# Autodesk Inventor assembly: Color Sorter
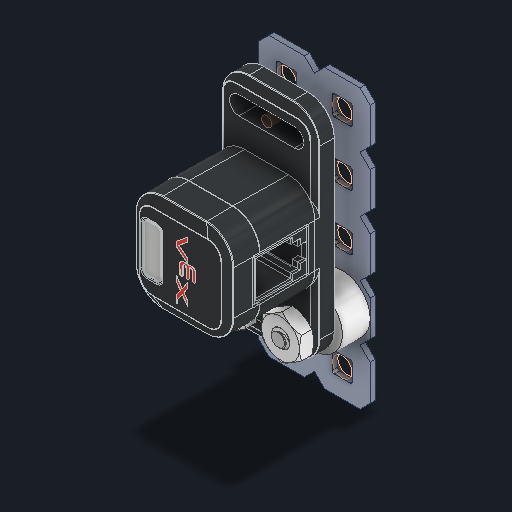
[picture p0: Inventor's stored thumbnail of the model, 512x512]
Saved by Autodesk Inventor 2025.1 (Build 291241000, 241)
## iProperties
Created: 2024-11-18
Part Number: Color Sorter
Document SubType Name: Assembly
Designer: avere
Author: avere
## Documents named in this file (8)
- C:\Users\avere\VEX\High Stakes\CAD\V3\Tower\Color Sorter.iam
- C:\Users\avere\VEX\High Stakes\CAD\ROBOPROS-CAD-Inventor\Electronics\Sensors\V5 Optical Sensor.ipt
- C:\Users\avere\VEX\High Stakes\CAD\ROBOPROS-CAD-Inventor\Structure\Plate\Steel\Steel Plate 2x5.ipt
- C:\Users\avere\VEX\High Stakes\CAD\ROBOPROS-CAD-Inventor\Motion\Spacers\Spacer Nylon .500 OD\NSpacer White .500 OD x .250.ipt
- C:\Users\avere\VEX\High Stakes\CAD\ROBOPROS-CAD-Inventor\Motion\Spacers\Spacer Nylon .500 OD.ipt
- C:\Users\avere\VEX\High Stakes\CAD\ROBOPROS-CAD-Inventor\Structure\Hardware\Screw Nylon - Pan Head\NScrew Pan Head Threaded .625.ipt
- C:\Users\avere\VEX\High Stakes\CAD\ROBOPROS-CAD-Inventor\Structure\Hardware\Nut Nylon\Nut Nylon - White.ipt
- C:\Users\avere\VEX\High Stakes\CAD\ROBOPROS-CAD-Inventor\Structure\Hardware\Nut Nylon.ipt
## Components (8 placed, 5 different names)
1. V5 Optical Sensor:1 — Insert:5
2. Steel Plate 2x5:1 — Insert:3, Insert:4
3. NSpacer White .500 OD x .250:1 — Insert:3
4. Nut Nylon - White:1 — Insert:5
5. NScrew Pan Head Threaded .625:1 — Insert:4
6. NSpacer White .500 OD x .250:2
7. Nut Nylon - White:2
8. NScrew Pan Head Threaded .625:2
## Component patterns: (2 elements, first: NSpacer White .500 OD x .250:1 + Nut Nylon - White:1 + NScrew Pan Head Threaded .625:1)
## Relationships (6: Insert 5, Mate 1)
- [Insert] (6.35 mm): V5 Optical Sensor:1 ↔ Steel Plate 2x5:1
- [Mate]: V5 Optical Sensor:1 ↔ Steel Plate 2x5:1
- [Insert]: V5 Optical Sensor:1 ↔ NSpacer White .500 OD x .250:1
- Insert:3: Steel Plate 2x5:1 ↔ NSpacer White .500 OD x .250:1
- Insert:4: Steel Plate 2x5:1 ↔ NScrew Pan Head Threaded .625:1
- Insert:5: V5 Optical Sensor:1 ↔ Nut Nylon - White:1
